# Autodesk Inventor assembly: Chassis Assembly
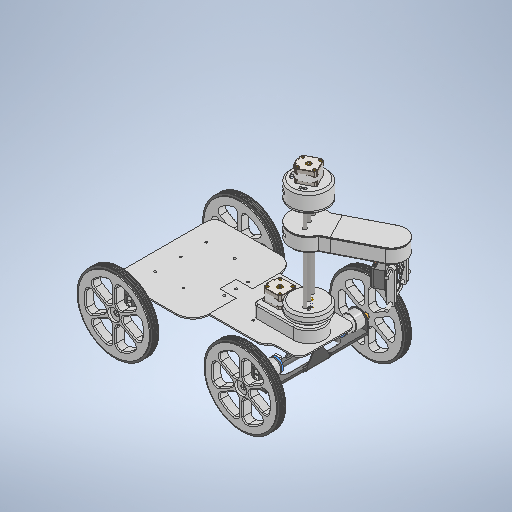
[picture p0: Inventor's stored thumbnail of the model, 512x512]
Saved by Autodesk Inventor 2025.2 (Build 292293000, 293)
## iProperties
Created: 2025-01-16
Part Number: Chassis Assembly
Document SubType Name: Assembly
Designer: Matt Tidd
Author: Matt Tidd
## Documents named in this file (8)
- C:\Users\mtidd2\Desktop\H2A\CAD\Chassis_Design\Chassis Assembly.iam
- C:\Users\mtidd2\Desktop\H2A\CAD\Motors_and_Wheels\Pendulum Suspension\Pendulum Suspension Assembly.iam
- C:\Users\mtidd2\Desktop\H2A\CAD\Motors_and_Wheels\Wheel Assembly\Motor Wheel Assembly.iam
- C:\Users\mtidd2\Desktop\H2A\CAD\Chassis_Design\Chassis Front Spine.ipt
- C:\Users\mtidd2\Desktop\H2A\CAD\Chassis_Design\Chassis Rear Spine 2.ipt
- C:\Users\mtidd2\Desktop\H2A\CAD\Chassis_Design\Chassis Rear Plate.ipt
- C:\Users\mtidd2\Desktop\H2A\CAD\Chassis_Design\Chassis Front Plate.ipt
- C:\Users\mtidd2\Desktop\H2A\CAD\SCARA\!SCARA assembly.iam
## Components (8 placed, 7 different names)
1. Motor Wheel Assembly:1 [sub-assembly] — Mate:3, Mate:9, Mate:10
2. Motor Wheel Assembly:2 [sub-assembly] — Mate:11, Mate:12, Mate:13
3. Pendulum Suspension Assembly:1 [sub-assembly] — Mate:2, Mate:7, Mate:8
4. Chassis Front Spine:1 — Mate:2, Mate:5, Mate:7, Mate:8
5. Chassis Rear Spine 2:1 — Mate:3, Mate:4, Mate:9, Mate:10, Mate:11, Mate:12, Mate:13
6. Chassis Rear Plate:1 — Mate:4
7. Chassis Front Plate:1 — Mate:5, Mate:6
8. !SCARA assembly:1 [sub-assembly] — Mate:6
## Relationships (12: Mate 12)
- Mate:2: Pendulum Suspension Assembly:1 ↔ Chassis Front Spine:1
- Mate:3: Motor Wheel Assembly:1 ↔ Chassis Rear Spine 2:1
- Mate:4: Chassis Rear Spine 2:1 ↔ Chassis Rear Plate:1
- Mate:5: Chassis Front Spine:1 ↔ Chassis Front Plate:1
- Mate:6: Chassis Front Plate:1 ↔ !SCARA assembly:1
- Mate:7: Pendulum Suspension Assembly:1 ↔ Chassis Front Spine:1
- Mate:8: Pendulum Suspension Assembly:1 ↔ Chassis Front Spine:1
- Mate:9: Motor Wheel Assembly:1 ↔ Chassis Rear Spine 2:1
- Mate:10: Motor Wheel Assembly:1 ↔ Chassis Rear Spine 2:1
- Mate:11: Motor Wheel Assembly:2 ↔ Chassis Rear Spine 2:1
- Mate:12: Motor Wheel Assembly:2 ↔ Chassis Rear Spine 2:1
- Mate:13: Motor Wheel Assembly:2 ↔ Chassis Rear Spine 2:1
